# Autodesk Inventor assembly: BoronProbe
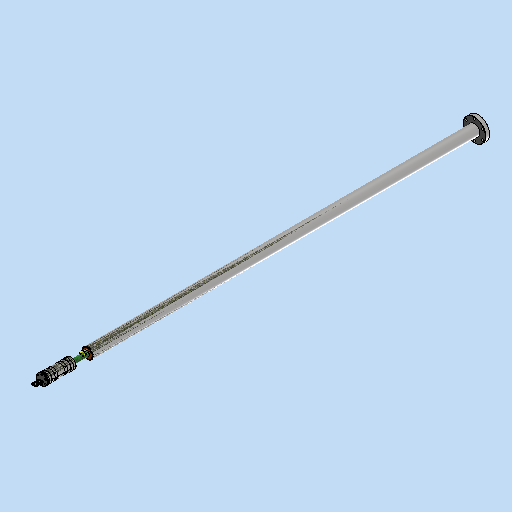
[picture p0: Inventor's stored thumbnail of the model, 512x512]
Saved by Autodesk Inventor 2025 (Build 290162000, 162)
## iProperties
Created: 2024-05-30
Part Number: BoronProbe
Document SubType Name: Assembly
Designer: kuzmin
Author: kuzmin
## Documents named in this file (10)
- C:\Users\queez\Dropbox\Drawings\PIHTI\BoronProbe\BoronProbe.iam
- C:\Users\queez\Dropbox\Drawings\PIHTI\PALP\CF34-nipples-for-PALP\ICF34_70mmNipple.iam
- C:\Users\queez\Dropbox\Drawings\PIHTI\PALP\Prototype-PALP-ring-to-pipe-adapter_4mm.ipt
- C:\Users\queez\Dropbox\Drawings\PIHTI\ContentCenter\Ceramics\Electric-feeds\feed_4.ipt
- C:\Users\queez\Dropbox\Drawings\PIHTI\PALP\Prototype-PALP-pipe-neck-straight.ipt
- C:\Users\queez\Dropbox\Drawings\PIHTI\PALP\Prototype-PALP-CF34-flange.ipt
- C:\Users\queez\Dropbox\Drawings\PIHTI\PALP\wire_connector.ipt
- C:\Users\queez\Dropbox\Drawings\PIHTI\PALP\Probe-clamp-v1.iam
- C:\Users\queez\Dropbox\Drawings\PIHTI\BoronProbe\BoronProbePipe.iam
- C:\Users\queez\Dropbox\Drawings\PIHTI\BoronProbe\BoronProbeHead.iam
## Components (12 placed, 9 different names)
1. BoronProbePipe:1 [sub-assembly]
2. ICF34_70mmNipple:1 [sub-assembly] — Rotational:2, Mate:4, Mate:15, Rigid:9
3. Prototype-PALP-ring-to-pipe-adapter_4mm:1 — Rotational:6, Flush:1, Rigid:7, Rigid:8
4. feed_4:1 — Cylindrical:1, Rigid:8
5. feed_4:2 — Cylindrical:2, Rigid:7
6. Prototype-PALP-pipe-neck-straight:1 — Rotational:6, Rigid:4
7. Prototype-PALP-CF34-flange:1 — Rigid:4, Rotational:2, Mate:4, Mate:5
8. wire_connector:1 — Cylindrical:1
9. wire_connector:2 — Cylindrical:2
10. Probe-clamp-v1:1 [sub-assembly] — Mate:16
11. Probe-clamp-v1:2 [sub-assembly] — Mate:15, Mate:16
12. BoronProbeHead:1 [sub-assembly] — Rigid:9
## Relationships (18: Mate 8, WeldJoint 4, RevoluteJoint 3, CylindricalJoint 2, Flush 1)
- [Mate]: BoronProbePipe:1 ↔ ICF34_70mmNipple:1
- [Mate]: BoronProbePipe:1 ↔ Prototype-PALP-ring-to-pipe-adapter_4mm:1
- [RevoluteJoint]: BoronProbePipe:1 ↔ Prototype-PALP-ring-to-pipe-adapter_4mm:1
- Rotational:6 [RevoluteJoint]: Prototype-PALP-ring-to-pipe-adapter_4mm:1 ↔ Prototype-PALP-pipe-neck-straight:1
- Rigid:4 [WeldJoint]: Prototype-PALP-pipe-neck-straight:1 ↔ Prototype-PALP-CF34-flange:1
- Rotational:2 [RevoluteJoint]: ICF34_70mmNipple:1 ↔ Prototype-PALP-CF34-flange:1
- Mate:4: ICF34_70mmNipple:1 ↔ Prototype-PALP-CF34-flange:1
- Flush:1: Prototype-PALP-ring-to-pipe-adapter_4mm:1
- Mate:5: Prototype-PALP-CF34-flange:1
- [Mate]: ICF34_70mmNipple:1 ↔ Probe-clamp-v1:1
- [Mate]: Probe-clamp-v1:1
- Cylindrical:1: feed_4:1 ↔ wire_connector:1
- Cylindrical:2: feed_4:2 ↔ wire_connector:2
- Rigid:7 [WeldJoint]: Prototype-PALP-ring-to-pipe-adapter_4mm:1 ↔ feed_4:2
- Rigid:8 [WeldJoint]: Prototype-PALP-ring-to-pipe-adapter_4mm:1 ↔ feed_4:1
- Mate:15: ICF34_70mmNipple:1 ↔ Probe-clamp-v1:2
- Mate:16: Probe-clamp-v1:1 ↔ Probe-clamp-v1:2
- Rigid:9 [WeldJoint]: ICF34_70mmNipple:1 ↔ BoronProbeHead:1
